# Autodesk Inventor assembly: gear40
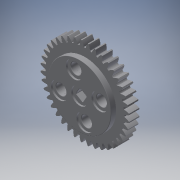
[picture p0: Inventor's stored thumbnail of the model, 180x180]
Saved by Autodesk Inventor 2019.3 (Build 233278000, 278)
## iProperties
Created: 2019-01-24
Part Number: gear40
Document SubType Name: Assembly
Designer: Varga Daniel
Author: Varga Daniel
## Documents named in this file (3)
- C:\!_Dani\!_cloud\OneDrive\!_munka\Revolution\RevvyDemoKit\Structural parts\Gears\gear40.iam
- C:\!_Dani\!_cloud\OneDrive\!_munka\Revolution\RevvyDemoKit\Structural parts\Gears\gear40.ipt
- C:\!_Dani\!_cloud\OneDrive\!_munka\Revolution\RevvyDemoKit\Structural parts\Gears\gear_collar.ipt
## Components (3 placed, 2 different names)
1. gear_collar:1 — Flush:1, Flush:2, Mate:1
2. gear40:1 — Mate:1, Mate:3
3. gear_collar:2 — Flush:1, Flush:2, Mate:3
## Relationships (4: Flush 2, Mate 2)
- Flush:1: gear_collar:1 ↔ gear_collar:2
- Flush:2: gear_collar:1 ↔ gear_collar:2
- Mate:1: gear_collar:1 ↔ gear40:1
- Mate:3: gear40:1 ↔ gear_collar:2
